# Autodesk Inventor assembly: ガイド輪部分
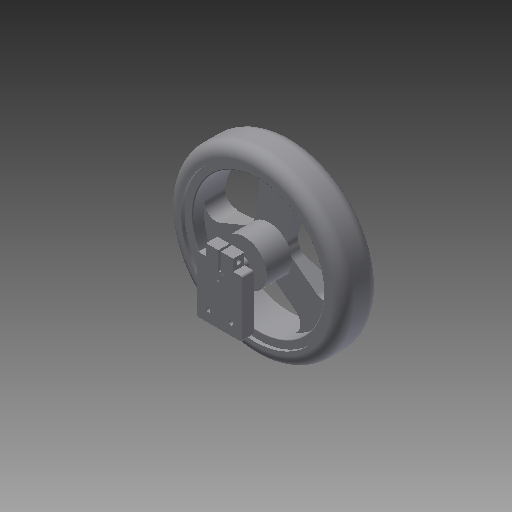
[picture p0: Inventor's stored thumbnail of the model, 512x512]
Saved by Autodesk Inventor 2017 (Build 210142000, 142)
## iProperties
Part Number: ガイド輪部分
Material: 一般
Document SubType Name: Assembly
Designer: highs
Author: highs
## Documents named in this file (4)
- C:\Users\highs\Desktop\学校\中の島\ガイド輪部分.iam
- C:\Users\highs\Desktop\学校\中の島\ガイド輪マウント.ipt
- C:\Users\highs\Desktop\学校\中の島\ガイド輪軸.ipt
- C:\Users\highs\Desktop\学校\中の島\ガイド輪.ipt
## Components (3 placed, 3 different names)
1. ガイド輪マウント:1 — メイト:1, フラッシュ:1, メイト:3
2. ガイド輪軸:1 — メイト:1, フラッシュ:1, メイト:2
3. ガイド輪:1 — メイト:2, メイト:3
## Relationships (4: Mate 3, Flush 1)
- メイト:1 [Mate]: ガイド輪マウント:1 ↔ ガイド輪軸:1
- フラッシュ:1 [Flush]: ガイド輪マウント:1 ↔ ガイド輪軸:1
- メイト:2 [Mate]: ガイド輪軸:1 ↔ ガイド輪:1
- メイト:3 [Mate] (12 mm): ガイド輪マウント:1 ↔ ガイド輪:1
